# Autodesk Inventor assembly: WingAssembly
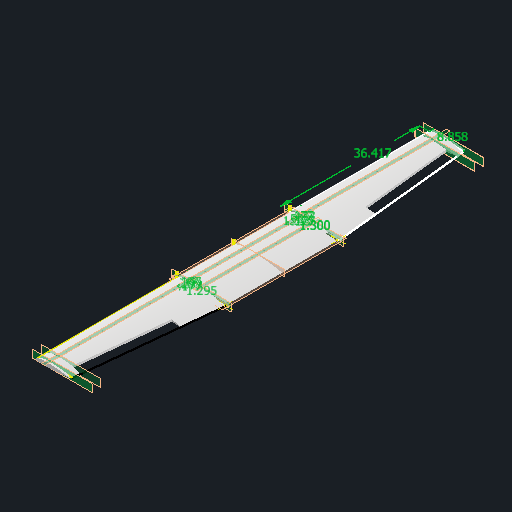
[picture p0: Inventor's stored thumbnail of the model, 512x512]
Saved by Autodesk Inventor 2026 (Build 300175050, 175E)
## iProperties
Created: 2025-06-04
Part Number: WingAssembly
Document SubType Name: Assembly
Designer: Cupri
Author: Cupri
## Documents named in this file (6)
- C:\Users\Cupri\OneDrive - University of South Carolina\Lab projects\UAV\SWIFT-UAV\System_development\Pelican\v0.2\SubAssemblies\WingAssembly\WingAssembly.iam
- C:\Users\Cupri\OneDrive - University of South Carolina\Lab projects\UAV\SWIFT-UAV\System_development\Pelican\v0.2\Parts\MiddleWing.ipt
- C:\Users\Cupri\OneDrive - University of South Carolina\Lab projects\UAV\SWIFT-UAV\System_development\Pelican\v0.2\Parts\OuterWingRight.ipt
- C:\Users\Cupri\OneDrive - University of South Carolina\Lab projects\UAV\SWIFT-UAV\System_development\Pelican\v0.2\Parts\OuterWingLeft.ipt
- C:\Users\Cupri\OneDrive - University of South Carolina\Lab projects\UAV\SWIFT-UAV\System_development\Pelican\v0.2\Parts\OuterWingRightCap.ipt
- C:\Users\Cupri\OneDrive - University of South Carolina\Lab projects\UAV\SWIFT-UAV\System_development\Pelican\v0.2\Parts\OuterWingRightCap_MIR.ipt
## Components (5 placed, 5 different names)
1. MiddleWing:1 — Mate:1, Flush:1, Rigid:1
2. OuterWingRight:1 — Mate:1, Flush:1, Rigid:1
3. OuterWingLeft:1
4. OuterWingRightCap:1
5. OuterWingRightCap_MIR:1
## Relationships (3: Mate 1, Flush 1, WeldJoint 1)
- Mate:1: MiddleWing:1 ↔ OuterWingRight:1
- Flush:1: MiddleWing:1 ↔ OuterWingRight:1
- Rigid:1 [WeldJoint]: MiddleWing:1 ↔ OuterWingRight:1
